# Autodesk Inventor assembly: endAssembly
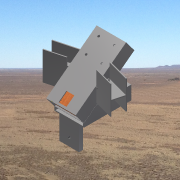
[picture p0: Inventor's stored thumbnail of the model, 180x180]
Saved by Autodesk Inventor 2014 SP1 (Build 180222100, 222)
## iProperties
Created: 2013-12-03
Part Number: endAssembly
Document SubType Name: Assembly
Designer: Dave
Author: Dave
## Documents named in this file (6)
- C:\Users\Dave\Desktop\hera-cad\support\endAssembly.iam
- C:\Users\Dave\Desktop\hera-cad\support\endHoriz.ipt
- C:\Users\Dave\Desktop\hera-cad\support\end37.ipt
- C:\Users\Dave\Desktop\hera-cad\support\endVert1.ipt
- C:\Users\Dave\Desktop\hera-cad\support\endVert1_MIR1.ipt
- C:\Users\Dave\Desktop\hera-cad\support\endWoodblock.ipt
## Components (5 placed, 5 different names)
1. endHoriz:1 — Mate:1, Flush:3, Flush:4, Flush:6
2. end37:1 — Mate:1, Flush:3, Mate:7, Mate:8, Mate:9, Mate:10
3. endVert1:1 — Mate:7, Flush:4, Flush:6
4. endVert1_MIR1:1
5. endWoodblock:1 — Mate:8, Mate:9, Mate:10
## Relationships (8: Mate 5, Flush 3)
- Mate:1: endHoriz:1 ↔ end37:1
- Flush:3: endHoriz:1 ↔ end37:1
- Mate:7: end37:1 ↔ endVert1:1
- Flush:4 (-50.8 mm): endHoriz:1 ↔ endVert1:1
- Flush:6 (38.1 mm): endHoriz:1 ↔ endVert1:1
- Mate:8: end37:1 ↔ endWoodblock:1
- Mate:9: end37:1 ↔ endWoodblock:1
- Mate:10: end37:1 ↔ endWoodblock:1
